# Autodesk Inventor assembly: ASY NDM-VOS_powder_hopper
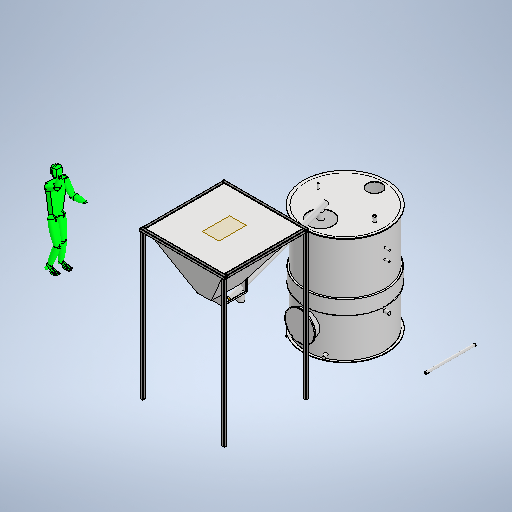
[picture p0: Inventor's stored thumbnail of the model, 512x512]
Saved by Autodesk Inventor 2025 (Build 290162010, 162A)
## iProperties
Created: 2024-07-24
Part Number: ASY NDM-VOS_powder_hopper
Document SubType Name: Assembly
Designer: admin
Author: admin
## Documents named in this file (9)
- C:\Users\admin\YandexDisk-badmisterfox\домашниий пк\Inventor\NDM-VOS_powder_hopper\ASY NDM-VOS_powder_hopper.iam
- C:\Users\admin\YandexDisk-badmisterfox\домашниий пк\Inventor\NDM-VOS_powder_hopper\Dummy 3.ipt
- C:\Users\admin\YandexDisk-badmisterfox\домашниий пк\Inventor\NDM-VOS_powder_hopper\NDM-VOS dummy2.ipt
- C:\Users\admin\YandexDisk-badmisterfox\домашниий пк\Inventor\NDM-VOS_powder_hopper\human 01\ч ASY human dummy 01.iam
- C:\Users\admin\YandexDisk-badmisterfox\домашниий пк\Inventor\NDM-VOS_powder_hopper\NDM-VOS dummy3.ipt
- C:\Users\admin\YandexDisk-badmisterfox\домашниий пк\Inventor\NDM-VOS_powder_hopper\Рама.iam
- C:\Users\admin\YandexDisk-badmisterfox\домашниий пк\Inventor\NDM-VOS_powder_hopper\NDM-VOS dummy4.ipt
- C:\Users\admin\YandexDisk-badmisterfox\домашниий пк\Inventor\NDM-VOS_powder_hopper\NDM-VOS dummy5.ipt
- C:\Users\admin\YandexDisk-badmisterfox\домашниий пк\Inventor\NDM-VOS_powder_hopper\NDM-VOS dummy6.ipt
## Components (9 placed, 8 different names)
1. NDM-VOS dummy3:1 — Flush:2, Flush:3, Flush:4, Rotational:1
2. Dummy 3:1 — Flush:1
3. NDM-VOS dummy2:1 — Flush:8, Mate:2
4. Рама:1 [sub-assembly] — Mate:1, Flush:5, Flush:6, Flush:8, Mate:2
5. NDM-VOS dummy4:1
6. NDM-VOS dummy4:2 — Rotational:1
7. NDM-VOS dummy5:1 — Flush:9, Mate:3
8. ч ASY human dummy 01:1 [sub-assembly]
9. NDM-VOS dummy6:1
## Relationships (12: Flush 8, Mate 3, RevoluteJoint 1)
- Flush:1: Dummy 3:1
- Flush:2: NDM-VOS dummy3:1
- Flush:3: NDM-VOS dummy3:1
- Flush:4: NDM-VOS dummy3:1
- Mate:1: Рама:1
- Flush:5 (800 mm): Рама:1
- Flush:6 (1600 mm): Рама:1
- Flush:8: NDM-VOS dummy2:1 ↔ Рама:1
- Mate:2: NDM-VOS dummy2:1 ↔ Рама:1
- Rotational:1 [RevoluteJoint]: NDM-VOS dummy3:1 ↔ NDM-VOS dummy4:2
- Flush:9: NDM-VOS dummy5:1
- Mate:3: NDM-VOS dummy5:1
